# Autodesk Inventor assembly: mounted-spool
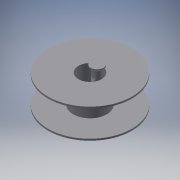
[picture p0: Inventor's stored thumbnail of the model, 180x180]
Saved by Autodesk Inventor 2018 (Build 220112000, 112)
## iProperties
Created: 2020-01-13
Part Number: mounted-spool
Document SubType Name: Assembly
Designer: Vinnie Caprarola
Author: Vinnie Caprarola
## Documents named in this file (3)
- Z:\Z\custom-parts\spool-mount\mounted-spool.iam
- Z:\Z\custom-parts\spool-mount\mount.ipt
- Z:\Z\custom-parts\spool-mount\spool.ipt
## Components (2 placed, 2 different names)
1. mount:1 — Tangent:1, Mate:1
2. spool:1 — Tangent:1, Mate:1
## Relationships (2: Tangent 1, Mate 1)
- Tangent:1: mount:1 ↔ spool:1
- Mate:1 (2 mm): mount:1 ↔ spool:1
